# Autodesk Inventor assembly: SimpleTHOR_v3
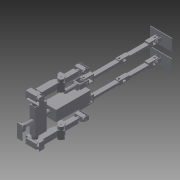
[picture p0: Inventor's stored thumbnail of the model, 180x180]
Saved by Autodesk Inventor 2013 (Build 170138000, 138)
## iProperties
Created: 2012-12-05
Part Number: SimpleTHOR_v3
Document SubType Name: Assembly
Designer: Joe
Author: Joe
## Documents named in this file (17)
- C:\Users\Joe\Dropbox\MyDocs\!RoMeLa\!RoMeLa Git\SimpleModel\Version2\SimpleTHOR_v3.iam
- C:\Users\Joe\Dropbox\MyDocs\!RoMeLa\!RoMeLa Git\SimpleModel\Version2\LowerTorso_v2.ipt
- C:\Users\Joe\Dropbox\MyDocs\!RoMeLa\!RoMeLa Git\SimpleModel\Version2\HipYaw_v2.ipt
- C:\Users\Joe\Dropbox\MyDocs\!RoMeLa\!RoMeLa Git\SimpleModel\Version2\HipRoll_v2.ipt
- C:\Users\Joe\Dropbox\MyDocs\!RoMeLa\!RoMeLa Git\SimpleModel\Version2\UpperLeg_v2.ipt
- C:\Users\Joe\Dropbox\MyDocs\!RoMeLa\!RoMeLa Git\SimpleModel\Version2\LowerLeg_v2.ipt
- C:\Users\Joe\Dropbox\MyDocs\!RoMeLa\!RoMeLa Git\SimpleModel\Version2\AnkRoll_v2.ipt
- C:\Users\Joe\Dropbox\MyDocs\!RoMeLa\!RoMeLa Git\SimpleModel\Version2\Foot.ipt
- C:\Users\Joe\Dropbox\MyDocs\!RoMeLa\!RoMeLa Git\SimpleModel\Version2\Neck_v2.ipt
- C:\Users\Joe\Dropbox\MyDocs\!RoMeLa\!RoMeLa Git\SimpleModel\Version2\Head_v2.ipt
- C:\Users\Joe\Dropbox\MyDocs\!RoMeLa\!RoMeLa Git\SimpleModel\Version2\NewArm\Sholder_Pitch.ipt
- C:\Users\Joe\Dropbox\MyDocs\!RoMeLa\!RoMeLa Git\SimpleModel\Version2\UpperTorso_v2.ipt
- C:\Users\Joe\Dropbox\MyDocs\!RoMeLa\!RoMeLa Git\SimpleModel\Version2\NewArm\Sholder_Roll.ipt
- C:\Users\Joe\Dropbox\MyDocs\!RoMeLa\!RoMeLa Git\SimpleModel\Version2\NewArm\Sholder_Yaw.ipt
- C:\Users\Joe\Dropbox\MyDocs\!RoMeLa\!RoMeLa Git\SimpleModel\Version2\NewArm\Elbow_Pitch.ipt
- C:\Users\Joe\Dropbox\MyDocs\!RoMeLa\!RoMeLa Git\SimpleModel\Version2\NewArm\Wrist_Yaw.ipt
- C:\Users\Joe\Dropbox\MyDocs\!RoMeLa\!RoMeLa Git\SimpleModel\Version2\NewArm\Wrist_Roll.ipt
## Components (28 placed, 28 different names)
1. torso — Mate:9, Mate:10, Mate:17, Mate:18
2. l_hip_yaw_mnt — Mate:53, Flush:12, Mate:54
3. l_hip_roll_mnt — Mate:53, Flush:12, Mate:54, Mate:55, Flush:13, Mate:56
4. l_thigh — Mate:5, Mate:6, Mate:55, Flush:13, Mate:56
5. l_shin — Mate:5, Mate:6
6. l_ankle_roll_mnt — Mate:57, Mate:58, Flush:14
7. l_ankle_pitch_mnt — Mate:57, Mate:58, Flush:14
8. r_hip_yaw_mnt — Mate:9, Mate:10, Mate:47, Mate:48, Flush:9
9. r_hip_roll_mnt — Mate:47, Mate:48, Flush:9, Mate:49, Mate:50, Flush:10
10. r_thigh — Mate:13, Mate:14, Mate:49, Mate:50, Flush:10
11. r_shin — Mate:13, Mate:14
12. r_ankle_roll_mnt — Mate:51, Mate:52, Flush:11
13. r_foot — Mate:51, Mate:52, Flush:11
14. chest — Mate:17, Mate:18, Mate:19, Mate:20, Mate:23, Mate:24, Mate:35, Mate:36
15. neck — Mate:19, Mate:20, Mate:21, Mate:22
16. head — Mate:21, Mate:22
17. l_sholder_pitch_mnt — Mate:23, Mate:24, Mate:25, Mate:26
18. l_sholder_roll_mnt — Mate:25, Mate:26, Mate:27, Mate:28
19. l_upper_arm — Mate:27, Mate:28, Mate:29, Mate:30
20. l_lower_arm — Mate:29, Mate:30, Mate:31, Mate:32
21. l_wrist — Mate:31, Mate:32, Mate:33, Mate:34
22. l_hand — Mate:33, Mate:34
23. r_sholder_pitch_mnt — Mate:35, Mate:36, Mate:37, Mate:38
24. r_sholder_roll_mnt — Mate:37, Mate:38, Mate:39, Mate:40
25. r_upper_arm — Mate:39, Mate:40, Mate:41, Mate:42
26. r_lower_arm — Mate:41, Mate:42, Mate:43, Mate:44
27. r_wrist — Mate:43, Mate:44, Mate:45, Mate:46
28. r_hand — Mate:45, Mate:46
## Relationships (54: Mate 48, Flush 6)
- Mate:5: l_thigh ↔ l_shin
- Mate:6: l_thigh ↔ l_shin
- Mate:9: torso ↔ r_hip_yaw_mnt
- Mate:10: torso ↔ r_hip_yaw_mnt
- Mate:13: r_thigh ↔ r_shin
- Mate:14: r_thigh ↔ r_shin
- Mate:17: torso ↔ chest
- Mate:18: torso ↔ chest
- Mate:19: chest ↔ neck
- Mate:20: chest ↔ neck
- Mate:21: neck ↔ head
- Mate:22: neck ↔ head
- Mate:23: chest ↔ l_sholder_pitch_mnt
- Mate:24: chest ↔ l_sholder_pitch_mnt
- Mate:25: l_sholder_pitch_mnt ↔ l_sholder_roll_mnt
- Mate:26: l_sholder_pitch_mnt ↔ l_sholder_roll_mnt
- Mate:27: l_sholder_roll_mnt ↔ l_upper_arm
- Mate:28: l_sholder_roll_mnt ↔ l_upper_arm
- Mate:29: l_upper_arm ↔ l_lower_arm
- Mate:30: l_upper_arm ↔ l_lower_arm
- Mate:31: l_lower_arm ↔ l_wrist
- Mate:32: l_lower_arm ↔ l_wrist
- Mate:33: l_wrist ↔ l_hand
- Mate:34: l_wrist ↔ l_hand
- Mate:35: chest ↔ r_sholder_pitch_mnt
- Mate:36: chest ↔ r_sholder_pitch_mnt
- Mate:37: r_sholder_pitch_mnt ↔ r_sholder_roll_mnt
- Mate:38: r_sholder_pitch_mnt ↔ r_sholder_roll_mnt
- Mate:39: r_sholder_roll_mnt ↔ r_upper_arm
- Mate:40: r_sholder_roll_mnt ↔ r_upper_arm
- Mate:41: r_upper_arm ↔ r_lower_arm
- Mate:42: r_upper_arm ↔ r_lower_arm
- Mate:43: r_lower_arm ↔ r_wrist
- Mate:44: r_lower_arm ↔ r_wrist
- Mate:45: r_wrist ↔ r_hand
- Mate:46: r_wrist ↔ r_hand
- Mate:47: r_hip_yaw_mnt ↔ r_hip_roll_mnt
- Mate:48: r_hip_yaw_mnt ↔ r_hip_roll_mnt
- Flush:9: r_hip_yaw_mnt ↔ r_hip_roll_mnt
- Mate:49: r_hip_roll_mnt ↔ r_thigh
- Mate:50: r_hip_roll_mnt ↔ r_thigh
- Flush:10: r_hip_roll_mnt ↔ r_thigh
- Mate:51: r_ankle_roll_mnt ↔ r_foot
- Mate:52: r_ankle_roll_mnt ↔ r_foot
- Flush:11: r_ankle_roll_mnt ↔ r_foot
- Mate:53: l_hip_yaw_mnt ↔ l_hip_roll_mnt
- Flush:12: l_hip_yaw_mnt ↔ l_hip_roll_mnt
- Mate:54: l_hip_yaw_mnt ↔ l_hip_roll_mnt
- Mate:55: l_hip_roll_mnt ↔ l_thigh
- Flush:13: l_hip_roll_mnt ↔ l_thigh
- Mate:56: l_hip_roll_mnt ↔ l_thigh
- Mate:57: l_ankle_roll_mnt ↔ l_ankle_pitch_mnt
- Mate:58: l_ankle_roll_mnt ↔ l_ankle_pitch_mnt
- Flush:14: l_ankle_roll_mnt ↔ l_ankle_pitch_mnt
